# Autodesk Inventor assembly: caseplegablepress
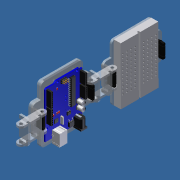
[picture p0: Inventor's stored thumbnail of the model, 180x180]
Saved by Autodesk Inventor 2014 (Build 180170000, 170)
## iProperties
Created: 2014-02-13
Part Number: caseplegablepress
Document SubType Name: Assembly
Designer: Lefo
Author: Lefo
## Documents named in this file (6)
- C:\Users\Lefo\Documents\Inventor\arduinoUno\pressfit\caseplegablepress.iam
- C:\Users\Lefo\Documents\Inventor\arduinoUno\arduino uno.iam
- C:\Users\Lefo\Documents\Inventor\arduinoUno\pressfit\baseProtoPress.iam
- C:\Users\Lefo\Documents\Inventor\arduinoUno\pressfit\linkpress.iam
- C:\Users\Lefo\Documents\Inventor\arduinoUno\pressfit\base2protopress.ipt
- C:\Users\Lefo\Documents\Inventor\arduinoUno\protoboard cortado.ipt
## Components (7 placed, 5 different names)
1. arduino uno:1 [sub-assembly] — Mate:1
2. baseProtoPress:1 [sub-assembly] — Mate:2
3. baseProtoPress:2 [sub-assembly] — Mate:1, Flush:1
4. base2protopress:1 — Flush:1
5. linkpress:1 [sub-assembly]
6. linkpress:2 [sub-assembly]
7. protoboard cortado:1 — Mate:2
## Relationships (3: Mate 2, Flush 1)
- Mate:1: arduino uno:1 ↔ baseProtoPress:2
- Flush:1: baseProtoPress:2 ↔ base2protopress:1
- Mate:2: baseProtoPress:1 ↔ protoboard cortado:1
